# Autodesk Inventor assembly: FilterWheel-Dynamixel(MX28)
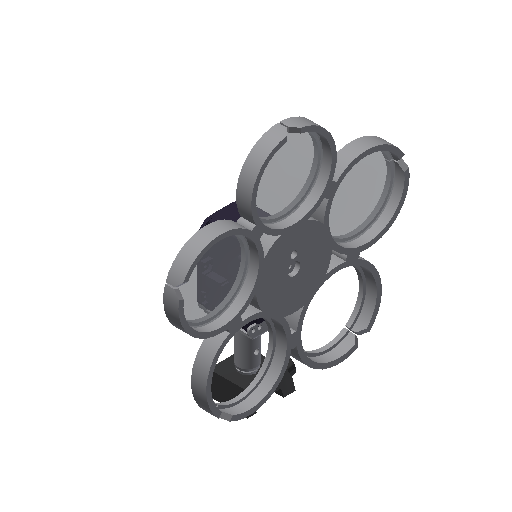
[picture p0: Inventor's stored thumbnail of the model, 512x512]
Saved by Autodesk Inventor 2023 (Build 270158000, 158)
## iProperties
Created: 2022-04-16
Part Number: FilterWheel-Dynamixel(MX28)
Document SubType Name: Assembly
Designer: Nikita
Author: Nikita
## Documents named in this file (7)
- C:\Users\Public\GitHub-public\benchtop-hardware\Benchtop\CAD-model-Inventor\mesoSPIM\detection_path\filter-wheel\FilterWheel-Dynamixel(MX28).iam
- C:\Users\Public\GitHub-public\benchtop-hardware\Benchtop\CAD-model-Inventor\library\Robotis\MX-28AT_AR.ipt
- C:\Users\Public\GitHub-public\benchtop-hardware\Benchtop\CAD-model-Inventor\library\Robotis\FR07-S101.ipt
- C:\Users\Public\GitHub-public\benchtop-hardware\Benchtop\custom-parts\deprecated\filter-wheel\FilterWheel-2inch-5pos.ipt
- C:\Users\Public\GitHub-public\benchtop-hardware\Benchtop\CAD-model-Inventor\library\Thorlabs\posts\12_7_mm_posts\TR30.ipt
- C:\Users\Public\GitHub-public\benchtop-hardware\Benchtop\CAD-model-Inventor\library\Thorlabs\rails\RC1.ipt
- C:\Users\Public\GitHub-public\benchtop-hardware\Benchtop\CAD-model-Inventor\mesoSPIM\detection_path\filter-wheel\Filter.ipt
## Components (8 placed, 6 different names)
1. MX-28AT_AR:1 — Mate:1, Insert:1, Angle:1, Insert:2
2. FR07-S101:1 — Mate:1, Insert:1, Angle:1, Insert:3
3. FilterWheel-2inch-5pos:1 — Insert:2, Angle:2
4. TR30:1 — Insert:3, Insert:4
5. RC1:1 — Insert:4, Angle:2
6. Filter:1
7. Filter:2
8. Filter:3
## Relationships (10: Insert 6, Angle 2, Mate 1, Flush 1)
- Mate:1: MX-28AT_AR:1 ↔ FR07-S101:1
- Insert:1: MX-28AT_AR:1 ↔ FR07-S101:1
- Angle:1 (0 deg): MX-28AT_AR:1 ↔ FR07-S101:1
- Insert:2: MX-28AT_AR:1 ↔ FilterWheel-2inch-5pos:1
- Insert:3: FR07-S101:1 ↔ TR30:1
- Insert:4: TR30:1 ↔ RC1:1
- Angle:2 (0 deg): FilterWheel-2inch-5pos:1 ↔ RC1:1
- [Flush]: FilterWheel-2inch-5pos:1 ↔ Filter:1
- [Insert]: FilterWheel-2inch-5pos:1 ↔ Filter:3
- [Insert]: FilterWheel-2inch-5pos:1 ↔ Filter:2
